# Autodesk Inventor assembly: Cart
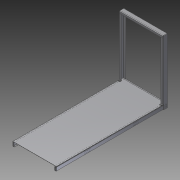
[picture p0: Inventor's stored thumbnail of the model, 180x180]
Saved by Autodesk Inventor 2012 (Build 160160000, 160)
## iProperties
Created: 2011-10-13
Part Number: Cart
Document SubType Name: Assembly
Designer: Tushar
Author: Tushar
## Documents named in this file (6)
- C:\Users\Tushar\Dropbox\CAD Inventor\Preseason Projects\Cart Competition Cart\Sah\Cart.iam
- C:\Users\Tushar\Dropbox\CAD Inventor\Preseason Projects\Cart Competition Cart\Sah\Base Side Bar.ipt
- C:\Users\Tushar\Dropbox\CAD Inventor\Preseason Projects\Cart Competition Cart\Sah\Base Back Bar.ipt
- C:\Users\Tushar\Dropbox\CAD Inventor\Preseason Projects\Cart Competition Cart\Sah\Base Top.ipt
- C:\Users\Tushar\Dropbox\CAD Inventor\Preseason Projects\Cart Competition Cart\Sah\Base Crossbar.ipt
- C:\Users\Tushar\Dropbox\CAD Inventor\Preseason Projects\Cart Competition Cart\Sah\Handle Bar.ipt
## Components (7 placed, 5 different names)
1. Base Side Bar:1 — Mate:1, Flush:1, Mate:2, Mate:9, Flush:5, Flush:6, Mate:11
2. Base Side Bar:2 — Mate:3, Mate:4, Flush:2, Mate:5, Mate:6, Mate:7, Mate:8, Flush:3, Flush:7
3. Base Back Bar:1 — Mate:1, Flush:1, Mate:2, Mate:3, Mate:4, Flush:2, Mate:10, Mate:12
4. Base Top:1 — Mate:9, Flush:5, Flush:6, Mate:13
5. Base Crossbar:1 — Mate:6, Mate:7, Flush:3
6. Base Crossbar:2 — Mate:5, Mate:8, Flush:7
7. Handle Bar:1 — Mate:10, Mate:11, Mate:12, Mate:13
## Relationships (19: Mate 13, Flush 6)
- Mate:1: Base Side Bar:1 ↔ Base Back Bar:1
- Flush:1: Base Side Bar:1 ↔ Base Back Bar:1
- Mate:2: Base Side Bar:1 ↔ Base Back Bar:1
- Mate:3: Base Side Bar:2 ↔ Base Back Bar:1
- Mate:4: Base Side Bar:2 ↔ Base Back Bar:1
- Flush:2: Base Side Bar:2 ↔ Base Back Bar:1
- Mate:5: Base Side Bar:2 ↔ Base Crossbar:2
- Mate:6: Base Side Bar:2 ↔ Base Crossbar:1
- Mate:7: Base Side Bar:2 ↔ Base Crossbar:1
- Mate:8: Base Side Bar:2 ↔ Base Crossbar:2
- Flush:3 (381 mm): Base Side Bar:2 ↔ Base Crossbar:1
- Mate:9: Base Side Bar:1 ↔ Base Top:1
- Flush:5: Base Side Bar:1 ↔ Base Top:1
- Flush:6: Base Side Bar:1 ↔ Base Top:1
- Mate:10: Base Back Bar:1 ↔ Handle Bar:1
- Mate:11: Base Side Bar:1 ↔ Handle Bar:1
- Mate:12: Base Back Bar:1 ↔ Handle Bar:1
- Mate:13: Base Top:1 ↔ Handle Bar:1
- Flush:7 (-381 mm): Base Side Bar:2 ↔ Base Crossbar:2
